# Autodesk Inventor assembly: Left Structure
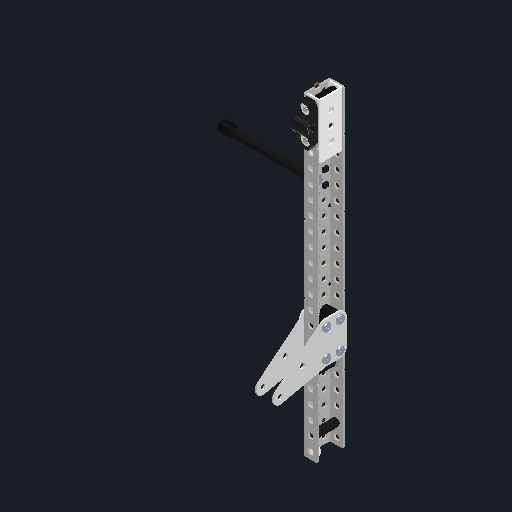
[picture p0: Inventor's stored thumbnail of the model, 512x512]
Saved by Autodesk Inventor 2025 (Build 290162000, 162)
## iProperties
Created: 2024-10-20
Part Number: Left Structure
Document SubType Name: Assembly
Designer: Averey Ku
Author: Averey Ku
## Documents named in this file (27)
- D:\VEX\High Stakes\CAD\V2\Tower\Left Structure.iam
- D:\VEX\High Stakes\CAD\ROBOPROS-CAD-Inventor\Structure\C Channel\Aluminum 1x2x1\Alu C 1x2x1x23.ipt
- D:\VEX\High Stakes\CAD\ROBOPROS-CAD-Inventor\Structure\Standoff\Standoff .75.ipt
- D:\VEX\High Stakes\CAD\ROBOPROS-CAD-Inventor\Motion\Spacers\Washer Steel\SWasher .375 OD x .062500.ipt
- D:\VEX\High Stakes\CAD\ROBOPROS-CAD-Inventor\Structure\Standoff\Standoff .875.ipt
- D:\VEX\High Stakes\CAD\ROBOPROS-CAD-Inventor\Structure\Hardware\Nut Nylon\Nut Nylon - White.ipt
- D:\VEX\High Stakes\CAD\ROBOPROS-CAD-Inventor\Motion\Shaft HS\HS Pillow Bearing Block.ipt
- D:\VEX\High Stakes\CAD\ROBOPROS-CAD-Inventor\Structure\Hardware\Screw Steel - Star\SScrew Star Smooth .290.ipt
- D:\VEX\High Stakes\CAD\ROBOPROS-CAD-Inventor\Structure\Hardware\Screw Shoulder Robosource\SScrew Shoulder Smooth .375 x .12.ipt
- D:\VEX\High Stakes\CAD\ROBOPROS-CAD-Inventor\Structure\Gussets\C Channel Coupler.ipt
- D:\VEX\High Stakes\CAD\ROBOPROS-CAD-Inventor\Motion\Spacers\Spacer Nylon .375 OD\NSpacer .375 OD x .250.ipt
- D:\VEX\High Stakes\CAD\ROBOPROS-CAD-Inventor\Motion\Spacers\Spacer Nylon .375 OD\NSpacer .375 OD x .500.ipt
- D:\VEX\High Stakes\CAD\ROBOPROS-CAD-Inventor\Structure\Hardware\Screw Steel - Star\SScrew Star Smooth 1.250.ipt
- D:\VEX\High Stakes\CAD\V2\Tower\Custom Parts\Angle Brace Gusset.ipt
- D:\VEX\High Stakes\CAD\ROBOPROS-CAD-Inventor\Structure\Standoff\Standoff .50.ipt
- D:\VEX\High Stakes\CAD\ROBOPROS-CAD-Inventor\Structure\Hardware\Screw Shoulder Robosource\SScrew Shoulder Smooth .290 x .09.ipt
- D:\VEX\High Stakes\CAD\ROBOPROS-CAD-Inventor\Structure\Hardware\Screw Shoulder Robosource\SScrew Shoulder Smooth .500 x .04.ipt
- D:\VEX\High Stakes\CAD\ROBOPROS-CAD-Inventor\Structure\Standoff\Standoff 3.00.ipt
- D:\VEX\High Stakes\CAD\ROBOPROS-CAD-Inventor\Structure\4-Post Standoff Retainer.ipt
- D:\VEX\High Stakes\CAD\ROBOPROS-CAD-Inventor\Structure\Hardware\Screw Steel - Star\SScrew Star Smooth .875.ipt
- D:\VEX\High Stakes\CAD\ROBOPROS-CAD-Inventor\Motion\Spacers\Spacer Nylon .375 OD\NSpacer .375 OD x .375.ipt
- C:\Users\avere\VEX\High Stakes\CAD\ROBOPROS-CAD-Inventor\Structure\Standoff.ipt
- C:\Users\avere\VEX\High Stakes\CAD\ROBOPROS-CAD-Inventor\Motion\Spacers\Washer Steel.ipt
- C:\Users\avere\VEX\High Stakes\CAD\ROBOPROS-CAD-Inventor\Structure\Hardware\Nut Nylon.ipt
- C:\Users\avere\VEX\High Stakes\CAD\ROBOPROS-CAD-Inventor\Structure\Hardware\Screw Steel - Star.ipt
- C:\Users\avere\VEX\High Stakes\CAD\ROBOPROS-CAD-Inventor\Structure\Hardware\Screw Shoulder Robosource.ipt
- C:\Users\avere\VEX\High Stakes\CAD\ROBOPROS-CAD-Inventor\Motion\Spacers\Spacer Nylon .375 OD.ipt
## Components (37 placed, 20 different names)
1. Alu C 1x2x1x23:1 — Mate:6
2. NSpacer .375 OD x .375:8 — Insert:32
3. Standoff .875:2
4. Nut Nylon - White:1
5. Standoff .75:1
6. SWasher .375 OD x .062500:1
7. SScrew Star Smooth .290:1
8. SScrew Shoulder Smooth .375 x .12:1
9. SScrew Star Smooth 1.250:3
10. HS Pillow Bearing Block:1
11. C Channel Coupler:1
12. Nut Nylon - White:2
13. Nut Nylon - White:3
14. NSpacer .375 OD x .250:1
15. NSpacer .375 OD x .500:2
16. NSpacer .375 OD x .250:3
17. NSpacer .375 OD x .500:4
18. SScrew Star Smooth 1.250:2
19. Angle Brace Gusset:1 — Insert:30
20. Angle Brace Gusset:2 — Insert:31
21. NSpacer .375 OD x .500:5
22. NSpacer .375 OD x .500:6
23. Standoff .50:3
24. NSpacer .375 OD x .500:7
25. SScrew Shoulder Smooth .375 x .12:2
26. SScrew Shoulder Smooth .290 x .09:3
27. SScrew Shoulder Smooth .500 x .04:4
28. Standoff 3.00:4 — Insert:32
29. 4-Post Standoff Retainer:1
30. Nut Nylon - White:4 — Insert:31
31. SScrew Star Smooth .875:4 — Insert:30
32. Nut Nylon - White:5
33. SScrew Star Smooth .875:5
34. Nut Nylon - White:6
35. SScrew Star Smooth .875:6
36. Nut Nylon - White:7
37. SScrew Star Smooth .875:7
## Component patterns: Gusset Mounting Hardware (4 elements)
## Relationships (36: Insert 30, Mate 6)
- [Insert]: Alu C 1x2x1x23:1 ↔ Standoff .75:1
- [Insert]: Standoff .75:1 ↔ SWasher .375 OD x .062500:1
- [Insert]: Alu C 1x2x1x23:1 ↔ Standoff .875:2
- [Insert]: Alu C 1x2x1x23:1 ↔ Nut Nylon - White:1
- [Insert]: Alu C 1x2x1x23:1 ↔ HS Pillow Bearing Block:1
- [Mate]: Alu C 1x2x1x23:1 ↔ HS Pillow Bearing Block:1
- [Insert]: Alu C 1x2x1x23:1 ↔ SScrew Star Smooth .290:1
- [Insert]: Alu C 1x2x1x23:1 ↔ SScrew Shoulder Smooth .375 x .12:1
- [Insert]: Alu C 1x2x1x23:1 ↔ C Channel Coupler:1
- [Mate]: Alu C 1x2x1x23:1 ↔ C Channel Coupler:1
- [Insert]: HS Pillow Bearing Block:1 ↔ Nut Nylon - White:3
- [Insert]: HS Pillow Bearing Block:1 ↔ Nut Nylon - White:2
- [Insert]: NSpacer .375 OD x .250:1 ↔ NSpacer .375 OD x .500:2
- [Insert]: C Channel Coupler:1 ↔ NSpacer .375 OD x .250:1
- [Insert]: NSpacer .375 OD x .250:3 ↔ NSpacer .375 OD x .500:4
- [Insert]: C Channel Coupler:1 ↔ NSpacer .375 OD x .500:4
- [Insert]: Alu C 1x2x1x23:1 ↔ SScrew Star Smooth 1.250:3
- [Insert]: Alu C 1x2x1x23:1 ↔ SScrew Star Smooth 1.250:2
- [Insert] (12.7 mm): Alu C 1x2x1x23:1 ↔ Angle Brace Gusset:1
- [Mate]: Alu C 1x2x1x23:1 ↔ Angle Brace Gusset:1
- [Insert]: Alu C 1x2x1x23:1 ↔ Angle Brace Gusset:2
- [Mate]: Alu C 1x2x1x23:1 ↔ Angle Brace Gusset:2
- [Insert]: Angle Brace Gusset:1 ↔ NSpacer .375 OD x .500:5
- [Insert]: Angle Brace Gusset:1 ↔ NSpacer .375 OD x .500:6
- [Insert]: Angle Brace Gusset:1 ↔ NSpacer .375 OD x .500:7
- [Insert]: Angle Brace Gusset:1 ↔ Standoff .50:3
- [Insert]: Angle Brace Gusset:2 ↔ SScrew Shoulder Smooth .375 x .12:2
- [Insert]: Angle Brace Gusset:1 ↔ SScrew Shoulder Smooth .290 x .09:3
- [Insert]: Alu C 1x2x1x23:1 ↔ SScrew Shoulder Smooth .500 x .04:4
- [Insert]: Alu C 1x2x1x23:1 ↔ 4-Post Standoff Retainer:1
- [Mate]: Alu C 1x2x1x23:1 ↔ 4-Post Standoff Retainer:1
- [Insert]: Standoff 3.00:4 ↔ 4-Post Standoff Retainer:1
- Mate:6: Alu C 1x2x1x23:1
- Insert:30: Angle Brace Gusset:1 ↔ SScrew Star Smooth .875:4
- Insert:31: Angle Brace Gusset:2 ↔ Nut Nylon - White:4
- Insert:32: NSpacer .375 OD x .375:8 ↔ Standoff 3.00:4
## Named parameters: d67_d65 = 0 mm
